# Autodesk Inventor assembly: NewChassis
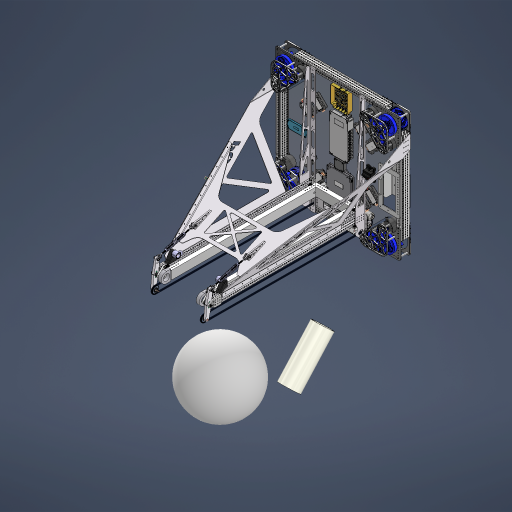
[picture p0: Inventor's stored thumbnail of the model, 512x512]
Saved by Autodesk Inventor 2024.3 (Build 283343000, 343)
## iProperties
ILogicPurgeVersion: 0.0.0.0
OnSaveVersion: 3.5.0.0
OnSaveAssembly: COREAutomationManager
Created: 2025-01-13
Part Number: NewChassis
Document SubType Name: Assembly
Designer: Marcus Tannini
Mfg Approved By: John.Thibert
Mass: 67130.1 g
Surface Area: 92907.1 cm^2
Volume: 47935.8 cm^3
Density: 1.40042 g/cm^3
ModelCat: Uncategorized
CN_MASS: 67.13
Author: Marcus Tannini
## Documents named in this file (43)
- \\clfs\homes\john.thibert\2025-Poseidon-Mechanical\#Poseidon 2025.iam
- \\clfs\homes\john.thibert\2025-Poseidon-Mechanical\ASSY,MK4i,Swerve_Module_INV.iam
- \\clfs\homes\john.thibert\2025-Poseidon-Mechanical\MAXTube-2x1-Holes.ipt
- \\clfs\homes\john.thibert\2025-Poseidon-Mechanical\BellyPanTop.ipt
- \\clfs\homes\john.thibert\2025-Poseidon-Mechanical\BellyPanBot.ipt
- \\clfs\homes\john.thibert\2025-Poseidon-Mechanical\BATTERY,12V.ipt
- \\clfs\homes\john.thibert\2025-Poseidon-Mechanical\CONTROLS,MAIN_BREAKER.ipt
- \\clfs\homes\john.thibert\2025-Poseidon-Mechanical\CONTROLS,MOTOR,NEO,550.ipt
- \\clfs\homes\john.thibert\2025-Poseidon-Mechanical\CONTROLS,PDH.ipt
- \\clfs\homes\john.thibert\2025-Poseidon-Mechanical\CONTROLS,PH.ipt
- \\clfs\homes\john.thibert\2025-Poseidon-Mechanical\CONTROLS,ROBO_RIO.ipt
- \\clfs\homes\john.thibert\2025-Poseidon-Mechanical\CONTROLS,SPARK_MAX.ipt
- \\clfs\homes\john.thibert\2025-Poseidon-Mechanical\CONTROLS,VRM.ipt
- \\clfs\homes\john.thibert\2025-Poseidon-Mechanical\COVER,SPARKMAX.ipt
- \\clfs\homes\john.thibert\2025-Poseidon-Mechanical\ModifiedCase(IncludesPatterning).iam
- \\clfs\homes\john.thibert\2025-Poseidon-Mechanical\PLATE,MOUNT,BATTERY,TOP.ipt
- \\clfs\homes\john.thibert\2025-Poseidon-Mechanical\PLATE,MOUNT,BATTERY,BOT.ipt
- \\clfs\homes\john.thibert\2025-Poseidon-Mechanical\MOUNT,STRAP,BATTERY.ipt
- \\clfs\homes\john.thibert\2025-Poseidon-Mechanical\SPACER,SPROCKET,IDLER,ELEVATOR.ipt
- \\clfs\homes\john.thibert\2025-Poseidon-Mechanical\22.ipt
- \\clfs\homes\john.thibert\2025-Poseidon-Mechanical\PLATE,MOUNT,DRIVE,ELEVATOR.ipt
- \\clfs\homes\john.thibert\2025-Poseidon-Mechanical\PLATE,BEARING,DRIVE,ELEVATOR.ipt
- \\clfs\homes\john.thibert\2025-Poseidon-Mechanical\PURCHASED,HEX_BEARING.ipt
- \\clfs\homes\john.thibert\2025-Poseidon-Mechanical\SHAFT,HEX,0.500in,DRIVE,ELEVATOR.ipt
- \\clfs\homes\john.thibert\2025-Poseidon-Mechanical\PLATE,SIDE,BRACE,RIGHT,ELEVATOR.ipt
- \\clfs\homes\john.thibert\2025-Poseidon-Mechanical\PLATE,SIDE,BRACE,LEFT,ELEVATOR.ipt
- \\clfs\homes\john.thibert\2025-Poseidon-Mechanical\PLATE,TURNBUCKLE,TENSIONER,CHAIN.ipt
- \\clfs\homes\john.thibert\2025-Poseidon-Mechanical\PLATE,BRACE,HORISONTAL,TOP,ELEVATOR.ipt
- \\clfs\homes\john.thibert\2025-Poseidon-Mechanical\TURNBUCKLE,0.25IN_CLEVIS.iam
- \\clfs\homes\john.thibert\2025-Poseidon-Mechanical\STAGE1,ELEVATOR.iam
- \\clfs\homes\john.thibert\2025-Poseidon-Mechanical\ASSY,MAIN,ELEVATOR.iam
- \\clfs\homes\john.thibert\2025-Poseidon-Mechanical\ANGLE,MOUNT,ELEVATOR.ipt
- \\clfs\homes\john.thibert\2025-Poseidon-Mechanical\ANGLE,MOUNT,ELEVATOR,MIRR.ipt
- \\clfs\homes\john.thibert\2025-Poseidon-Mechanical\FABRIC,BUMPERS.ipt
- \\clfs\homes\john.thibert\2025-Poseidon-Mechanical\9293K119_Constant-Force Spring.ipt
- \\clfs\homes\john.thibert\2025-Poseidon-Mechanical\MOUNT,SPRING,ELEVATOR.ipt
- \\clfs\homes\john.thibert\2025-Poseidon-Mechanical\MOUNT,SPRING,ELEVATOR,MIRR.ipt
- \\clfs\homes\john.thibert\2025-Poseidon-Mechanical\VersaPlanetary v2 Dual Stage 10_1 with RS 550 (1).iam
- \\clfs\homes\john.thibert\2025-Poseidon-Mechanical\CORAL.ipt
- \\clfs\homes\john.thibert\2025-Poseidon-Mechanical\algae.ipt
- \\clfs\homes\john.thibert\2025-Poseidon-Mechanical\BRACE,SHAFT,ELEVATOR.ipt
- \\clfs\homes\john.thibert\2025-Poseidon-Mechanical\WCP-0754.ipt
- \\clfs\homes\john.thibert\2025-Poseidon-Mechanical\SPACER,HEX,0.125IN.ipt
## Components (89 placed, 45 different names)
1. FABRIC,BUMPERS.ipt:1 — Flush:323, Mate:335, Mate:336
2. CORAL:1
3. algae:1
4. BellyPanBot.ipt:1 — Mate:66, Mate:353, Mate:354
5. BellyPanTop.ipt:1 — Mate:62, Mate:63, Mate:65, Mate:70, Mate:71, Mate:82, Mate:84, Insert:7, Insert:8, Insert:9, Insert:10, Insert:11, Insert:12, Insert:13, Insert:14, Insert:15, Insert:16, Insert:17, Insert:18, Insert:19, Insert:20, Insert:21, Insert:22, Mate:111, Mate:113, Mate:114, Mate:116, Mate:117, Mate:118, Mate:119, Mate:121, Mate:122, Mate:123, Mate:124, Mate:125, Mate:126, Mate:127, Mate:130, Insert:23, Insert:24, Mate:223, Mate:308, Mate:320, Mate:349, Mate:350
6. MAXTube-2x1-Holes.ipt:1 — Mate:1, Mate:2, Mate:3, Mate:4, Mate:5, Mate:15, Mate:115, Mate:272
7. MAXTube-2x1-Holes.ipt:2 — Mate:6, Mate:7, Mate:8, Mate:9, Mate:10, Mate:11, Mate:62, Mate:309, Mate:310
8. MAXTube-2x1-Holes.ipt:3 — Mate:19, Mate:20, Mate:21, Mate:66, Mate:114, Mate:312, Mate:313, Mate:336
9. MAXTube-2x1-Holes.ipt:4 — Mate:12, Mate:13, Mate:14, Mate:16, Mate:17, Mate:18, Mate:29, Mate:63, Mate:271, Mate:353, Mate:354
10. MOUNT,STRAP,BATTERY.ipt:1 — Mate:357, Mate:358, Mate:359
11. PLATE,MOUNT,BATTERY,BOT.ipt:1 — Mate:320, Mate:321, Mate:351, Mate:352
12. PLATE,MOUNT,BATTERY,TOP.ipt:1 — Mate:127, Mate:349, Mate:350, Mate:351, Mate:352, Mate:356, Mate:357, Mate:358, Mate:359
13. BATTERY,12V.ipt:1 — Mate:321, Mate:356
14. CONTROLS,MAIN_BREAKER.ipt:1 — Mate:82, Mate:111, Mate:116
15. CONTROLS,MOTOR,NEO,550.ipt:1
16. CONTROLS,PDH.ipt:1 — Mate:113, Mate:117, Mate:118, Mate:119
17. CONTROLS,PH.ipt:1 — Insert:23, Insert:24
18. CONTROLS,ROBO_RIO.ipt:1 — Mate:124, Mate:125, Mate:126
19. CONTROLS,SPARK_MAX.ipt:1 — Mate:84, Mate:85, Mate:86, Mate:87
20. CONTROLS,VRM.ipt:1 — Mate:121, Mate:122, Mate:123
21. ModifiedCase(IncludesPatterning).iam:1 [sub-assembly] — Mate:130
22. BRACE,SHAFT,ELEVATOR:1 — Mate:547, Mate:548, Insert:52, Insert:53, Mate:551, Mate:559
23. PURCHASED,HEX_BEARING:3 — Insert:53, Mate:549, Mate:557
24. PURCHASED,HEX_BEARING:4 — Insert:52, Mate:558
25. BRACE,SHAFT,ELEVATOR:2 — Mate:550, Mate:551, Mate:576
26. PURCHASED,HEX_BEARING:5
27. PURCHASED,HEX_BEARING:6 — Mate:555
28. 22:3 — Mate:552, Flush:331, Mate:555, Mate:560
29. WCP-0754:1 — Mate:553, Flush:331
30. SPACER,HEX,0.125IN:1 — Mate:556, Mate:557
31. SPACER,HEX,0.125IN:2 — Mate:558, Mate:559, Mate:560
32. BRACE,SHAFT,ELEVATOR:3 — Mate:565, Mate:568, Mate:569, Mate:576
33. PURCHASED,HEX_BEARING:7 — Mate:575
34. PURCHASED,HEX_BEARING:8
35. BRACE,SHAFT,ELEVATOR:4 — Mate:567, Mate:572, Mate:573
36. PURCHASED,HEX_BEARING:9 — Mate:570, Mate:574
37. PURCHASED,HEX_BEARING:10 — Mate:564
38. 22:4 — Mate:572
39. WCP-0754:2 — Mate:571, Mate:573, Mate:575
40. SPACER,HEX,0.125IN:3 — Mate:569, Mate:570, Mate:571
41. SPACER,HEX,0.125IN:4 — Mate:564, Mate:565
42. 22.ipt:1 — Mate:227, Angle:6
43. 22.ipt:2 — Mate:233, Angle:4, Flush:14
44. 9293K119_Constant-Force Spring:1 — Mate:364, Mate:365
45. 9293K119_Constant-Force Spring:2 — Mate:370, Mate:371
46. ANGLE,MOUNT,ELEVATOR,MIRR.ipt:1 — Mate:308, Mate:309, Mate:310, Mate:311, Mate:312, Mate:313, Mate:314, Mate:315, Flush:329
47. ANGLE,MOUNT,ELEVATOR.ipt:1 — Mate:65, Mate:70, Mate:71, Mate:161, Mate:162, Mate:224, STAGE1 LOWER LIMIT, STAGE1 MIN
48. ASSY,MAIN,ELEVATOR.iam:1 [sub-assembly] — Mate:161, Mate:162, Flush:19, Mate:297, STAGE1 UPPER LIMIT, STAGE1 MAX, Mate:311, Mate:314, Mate:315, Mate:363, Mate:362, Mate:366, Mate:367, Mate:368, Mate:369, Mate:548, Mate:552
49. CONTROLS,MOTOR,NEO,550:3
50. CONTROLS,MOTOR,NEO,550:4
51. MOUNT,SPRING,ELEVATOR,MIRR:1 — Mate:367, Mate:368, Mate:369, Mate:370, Mate:371
52. MOUNT,SPRING,ELEVATOR:1 — Mate:363, Mate:362, Mate:364, Mate:365, Mate:366
53. PLATE,BEARING,DRIVE,ELEVATOR.ipt:1 — Mate:226, Mate:227, Mate:228, Mate:229, Insert:50
54. PLATE,BEARING,DRIVE,ELEVATOR.ipt:2 — Mate:230, Mate:231, Mate:232, Insert:49, Mate:233, Mate:234
55. PLATE,BRACE,HORISONTAL,TOP,ELEVATOR.ipt:1 — Mate:285, Mate:286, Mate:289, Mate:290, Mate:291, Mate:295, Mate:296
56. PLATE,MOUNT,DRIVE,ELEVATOR.ipt:1 — Mate:223, Mate:224, Mate:226, Mate:228, Mate:229, Mate:230, Mate:231, Mate:232, Flush:329, Mate:469, Mate:470, Mate:471, Mate:472, Mate:473, Mate:474
57. PLATE,SIDE,BRACE,LEFT,ELEVATOR.ipt:1 — Mate:271, Mate:289, Mate:290, Mate:291, Mate:335
58. PLATE,SIDE,BRACE,RIGHT,ELEVATOR.ipt:1 — Mate:272
59. PLATE,TURNBUCKLE,TENSIONER,CHAIN.ipt:1 — Mate:285, Mate:296
60. PLATE,TURNBUCKLE,TENSIONER,CHAIN.ipt:2 — Mate:286, Mate:295
61. PURCHASED,HEX_BEARING.ipt:1 — Insert:49, Angle:5
62. PURCHASED,HEX_BEARING.ipt:2 — Insert:50, Angle:7
63. SHAFT,HEX,0.500in,DRIVE,ELEVATOR.ipt:1 — Mate:234, Angle:4, Angle:5, Angle:6, Angle:7, Flush:14
64. SPACER,SPROCKET,IDLER,ELEVATOR.ipt:1
65. SPACER,SPROCKET,IDLER,ELEVATOR.ipt:2
66. STAGE1,ELEVATOR.iam:1 [sub-assembly] — Flush:19, Mate:297, STAGE1 LOWER LIMIT, STAGE1 UPPER LIMIT, STAGE1 MIN, STAGE1 MAX
67. TURNBUCKLE,0.25IN_CLEVIS.iam:1 [sub-assembly]
68. TURNBUCKLE,0.25IN_CLEVIS.iam:2 [sub-assembly]
69. VersaPlanetary v2 Dual Stage 10_1 with RS 550 (1):1 [sub-assembly] — Mate:472, Mate:473, Mate:474, Mate:547, Mate:549, Mate:550, Mate:553, Mate:556
70. VersaPlanetary v2 Dual Stage 10_1 with RS 550 (1):2 [sub-assembly] — Mate:469, Mate:470, Mate:471, Mate:567, Mate:568, Mate:574
71. ASSY,MK4i,Swerve_Module_INV.iam:1 [sub-assembly] — Mate:1, Mate:2, Mate:15
72. ASSY,MK4i,Swerve_Module_INV.iam:2 [sub-assembly] — Mate:3, Mate:4, Mate:5, Mate:6, Mate:7, Mate:8
73. ASSY,MK4i,Swerve_Module_INV.iam:3 [sub-assembly] — Mate:9, Mate:10, Mate:11, Mate:12, Mate:13, Mate:14
74. ASSY,MK4i,Swerve_Module_INV.iam:4 [sub-assembly] — Mate:16, Mate:17, Mate:18, Mate:19, Mate:20, Mate:21, Mate:67
75. CONTROLS,SPARK_MAX.ipt:2
76. CONTROLS,SPARK_MAX.ipt:3
77. CONTROLS,SPARK_MAX.ipt:4
78. CONTROLS,SPARK_MAX.ipt:5
79. CONTROLS,SPARK_MAX.ipt:6
80. CONTROLS,SPARK_MAX.ipt:7
81. CONTROLS,SPARK_MAX.ipt:8
82. COVER,SPARKMAX.ipt:1 — Mate:85, Mate:86, Mate:87, Insert:7, Insert:8
83. COVER,SPARKMAX.ipt:2 — Insert:9, Insert:10
84. COVER,SPARKMAX.ipt:3 — Insert:11, Insert:12
85. COVER,SPARKMAX.ipt:4 — Insert:13, Insert:14
86. COVER,SPARKMAX.ipt:5 — Insert:17, Insert:18
87. COVER,SPARKMAX.ipt:6 — Insert:15, Insert:16
88. COVER,SPARKMAX.ipt:7 — Insert:21, Insert:22
89. COVER,SPARKMAX.ipt:8 — Insert:19, Insert:20
## Relationships (224: Mate 180, Insert 32, Flush 8, Angle 4)
- Mate:1: MAXTube-2x1-Holes.ipt:1 ↔ ASSY,MK4i,Swerve_Module_INV.iam:1
- Mate:2: MAXTube-2x1-Holes.ipt:1 ↔ ASSY,MK4i,Swerve_Module_INV.iam:1
- Mate:3: MAXTube-2x1-Holes.ipt:1 ↔ ASSY,MK4i,Swerve_Module_INV.iam:2
- Mate:4: MAXTube-2x1-Holes.ipt:1 ↔ ASSY,MK4i,Swerve_Module_INV.iam:2
- Mate:5: MAXTube-2x1-Holes.ipt:1 ↔ ASSY,MK4i,Swerve_Module_INV.iam:2
- Mate:6: MAXTube-2x1-Holes.ipt:2 ↔ ASSY,MK4i,Swerve_Module_INV.iam:2
- Mate:7: MAXTube-2x1-Holes.ipt:2 ↔ ASSY,MK4i,Swerve_Module_INV.iam:2
- Mate:8: MAXTube-2x1-Holes.ipt:2 ↔ ASSY,MK4i,Swerve_Module_INV.iam:2
- Mate:9: MAXTube-2x1-Holes.ipt:2 ↔ ASSY,MK4i,Swerve_Module_INV.iam:3
- Mate:10: MAXTube-2x1-Holes.ipt:2 ↔ ASSY,MK4i,Swerve_Module_INV.iam:3
- Mate:11: MAXTube-2x1-Holes.ipt:2 ↔ ASSY,MK4i,Swerve_Module_INV.iam:3
- Mate:12: MAXTube-2x1-Holes.ipt:4 ↔ ASSY,MK4i,Swerve_Module_INV.iam:3
- Mate:13: MAXTube-2x1-Holes.ipt:4 ↔ ASSY,MK4i,Swerve_Module_INV.iam:3
- Mate:14: MAXTube-2x1-Holes.ipt:4 ↔ ASSY,MK4i,Swerve_Module_INV.iam:3
- Mate:15: MAXTube-2x1-Holes.ipt:1 ↔ ASSY,MK4i,Swerve_Module_INV.iam:1
- Mate:16: MAXTube-2x1-Holes.ipt:4 ↔ ASSY,MK4i,Swerve_Module_INV.iam:4
- Mate:17: MAXTube-2x1-Holes.ipt:4 ↔ ASSY,MK4i,Swerve_Module_INV.iam:4
- Mate:18: MAXTube-2x1-Holes.ipt:4 ↔ ASSY,MK4i,Swerve_Module_INV.iam:4
- Mate:19: MAXTube-2x1-Holes.ipt:3 ↔ ASSY,MK4i,Swerve_Module_INV.iam:4
- Mate:20: MAXTube-2x1-Holes.ipt:3 ↔ ASSY,MK4i,Swerve_Module_INV.iam:4
- Mate:21: MAXTube-2x1-Holes.ipt:3 ↔ ASSY,MK4i,Swerve_Module_INV.iam:4
- Mate:29 (-6.35 mm): MAXTube-2x1-Holes.ipt:4
- Mate:62: BellyPanTop.ipt:1 ↔ MAXTube-2x1-Holes.ipt:2
- Mate:63: BellyPanTop.ipt:1 ↔ MAXTube-2x1-Holes.ipt:4
- Mate:65: BellyPanTop.ipt:1 ↔ ANGLE,MOUNT,ELEVATOR.ipt:1
- Mate:66: BellyPanBot.ipt:1 ↔ MAXTube-2x1-Holes.ipt:3
- Mate:67 (35.56 mm): ASSY,MK4i,Swerve_Module_INV.iam:4
- Mate:70: BellyPanTop.ipt:1 ↔ ANGLE,MOUNT,ELEVATOR.ipt:1
- Mate:71: BellyPanTop.ipt:1 ↔ ANGLE,MOUNT,ELEVATOR.ipt:1
- Mate:321: PLATE,MOUNT,BATTERY,BOT.ipt:1 ↔ BATTERY,12V.ipt:1
- Mate:82: BellyPanTop.ipt:1 ↔ CONTROLS,MAIN_BREAKER.ipt:1
- Mate:84: BellyPanTop.ipt:1 ↔ CONTROLS,SPARK_MAX.ipt:1
- Mate:85: CONTROLS,SPARK_MAX.ipt:1 ↔ COVER,SPARKMAX.ipt:1
- Mate:86: CONTROLS,SPARK_MAX.ipt:1 ↔ COVER,SPARKMAX.ipt:1
- Mate:87: CONTROLS,SPARK_MAX.ipt:1 ↔ COVER,SPARKMAX.ipt:1
- Insert:7: BellyPanTop.ipt:1 ↔ COVER,SPARKMAX.ipt:1
- Insert:8: BellyPanTop.ipt:1 ↔ COVER,SPARKMAX.ipt:1
- [Mate]: CONTROLS,SPARK_MAX.ipt:2 ↔ COVER,SPARKMAX.ipt:2
- [Mate]: CONTROLS,SPARK_MAX.ipt:2 ↔ COVER,SPARKMAX.ipt:2
- [Mate]: CONTROLS,SPARK_MAX.ipt:2 ↔ COVER,SPARKMAX.ipt:2
- [Mate]: CONTROLS,SPARK_MAX.ipt:3 ↔ COVER,SPARKMAX.ipt:3
- [Mate]: CONTROLS,SPARK_MAX.ipt:3 ↔ COVER,SPARKMAX.ipt:3
- [Mate]: CONTROLS,SPARK_MAX.ipt:3 ↔ COVER,SPARKMAX.ipt:3
- [Mate]: CONTROLS,SPARK_MAX.ipt:4 ↔ COVER,SPARKMAX.ipt:4
- [Mate]: CONTROLS,SPARK_MAX.ipt:4 ↔ COVER,SPARKMAX.ipt:4
- [Mate]: CONTROLS,SPARK_MAX.ipt:4 ↔ COVER,SPARKMAX.ipt:4
- [Mate]: CONTROLS,SPARK_MAX.ipt:5 ↔ COVER,SPARKMAX.ipt:5
- [Mate]: CONTROLS,SPARK_MAX.ipt:5 ↔ COVER,SPARKMAX.ipt:5
- [Mate]: CONTROLS,SPARK_MAX.ipt:5 ↔ COVER,SPARKMAX.ipt:5
- [Mate]: CONTROLS,SPARK_MAX.ipt:6 ↔ COVER,SPARKMAX.ipt:6
- [Mate]: CONTROLS,SPARK_MAX.ipt:6 ↔ COVER,SPARKMAX.ipt:6
- [Mate]: CONTROLS,SPARK_MAX.ipt:6 ↔ COVER,SPARKMAX.ipt:6
- [Mate]: CONTROLS,SPARK_MAX.ipt:7 ↔ COVER,SPARKMAX.ipt:7
- [Mate]: CONTROLS,SPARK_MAX.ipt:7 ↔ COVER,SPARKMAX.ipt:7
- [Mate]: CONTROLS,SPARK_MAX.ipt:7 ↔ COVER,SPARKMAX.ipt:7
- [Mate]: CONTROLS,SPARK_MAX.ipt:8 ↔ COVER,SPARKMAX.ipt:8
- [Mate]: CONTROLS,SPARK_MAX.ipt:8 ↔ COVER,SPARKMAX.ipt:8
- [Mate]: CONTROLS,SPARK_MAX.ipt:8 ↔ COVER,SPARKMAX.ipt:8
- Insert:9: BellyPanTop.ipt:1 ↔ COVER,SPARKMAX.ipt:2
- Insert:10: BellyPanTop.ipt:1 ↔ COVER,SPARKMAX.ipt:2
- Insert:11: BellyPanTop.ipt:1 ↔ COVER,SPARKMAX.ipt:3
- Insert:12: BellyPanTop.ipt:1 ↔ COVER,SPARKMAX.ipt:3
- Insert:13: BellyPanTop.ipt:1 ↔ COVER,SPARKMAX.ipt:4
- Insert:14: BellyPanTop.ipt:1 ↔ COVER,SPARKMAX.ipt:4
- Insert:15: BellyPanTop.ipt:1 ↔ COVER,SPARKMAX.ipt:6
- Insert:16: BellyPanTop.ipt:1 ↔ COVER,SPARKMAX.ipt:6
- Insert:17: BellyPanTop.ipt:1 ↔ COVER,SPARKMAX.ipt:5
- Insert:18: BellyPanTop.ipt:1 ↔ COVER,SPARKMAX.ipt:5
- Insert:19: BellyPanTop.ipt:1 ↔ COVER,SPARKMAX.ipt:8
- Insert:20: BellyPanTop.ipt:1 ↔ COVER,SPARKMAX.ipt:8
- Insert:21: BellyPanTop.ipt:1 ↔ COVER,SPARKMAX.ipt:7
- Insert:22: BellyPanTop.ipt:1 ↔ COVER,SPARKMAX.ipt:7
- Mate:111: BellyPanTop.ipt:1 ↔ CONTROLS,MAIN_BREAKER.ipt:1
- Mate:113: BellyPanTop.ipt:1 ↔ CONTROLS,PDH.ipt:1
- Mate:114: BellyPanTop.ipt:1 ↔ MAXTube-2x1-Holes.ipt:3
- Mate:115 (-374.65 mm): MAXTube-2x1-Holes.ipt:1
- Mate:116 (0.254 mm): BellyPanTop.ipt:1 ↔ CONTROLS,MAIN_BREAKER.ipt:1
- Mate:117: BellyPanTop.ipt:1 ↔ CONTROLS,PDH.ipt:1
- Mate:118: BellyPanTop.ipt:1 ↔ CONTROLS,PDH.ipt:1
- Mate:119: BellyPanTop.ipt:1 ↔ CONTROLS,PDH.ipt:1
- Mate:121: BellyPanTop.ipt:1 ↔ CONTROLS,VRM.ipt:1
- Mate:122: BellyPanTop.ipt:1 ↔ CONTROLS,VRM.ipt:1
- Mate:123: BellyPanTop.ipt:1 ↔ CONTROLS,VRM.ipt:1
- Mate:124: BellyPanTop.ipt:1 ↔ CONTROLS,ROBO_RIO.ipt:1
- Mate:125: BellyPanTop.ipt:1 ↔ CONTROLS,ROBO_RIO.ipt:1
- Mate:126: BellyPanTop.ipt:1 ↔ CONTROLS,ROBO_RIO.ipt:1
- Mate:127: BellyPanTop.ipt:1 ↔ PLATE,MOUNT,BATTERY,TOP.ipt:1
- Mate:130: BellyPanTop.ipt:1 ↔ ModifiedCase(IncludesPatterning).iam:1
- Insert:23: BellyPanTop.ipt:1 ↔ CONTROLS,PH.ipt:1
- Insert:24: BellyPanTop.ipt:1 ↔ CONTROLS,PH.ipt:1
- Mate:161: ANGLE,MOUNT,ELEVATOR.ipt:1 ↔ ASSY,MAIN,ELEVATOR.iam:1
- Mate:162: ANGLE,MOUNT,ELEVATOR.ipt:1 ↔ ASSY,MAIN,ELEVATOR.iam:1
- [Mate]: ANGLE,MOUNT,ELEVATOR.ipt:1 ↔ ASSY,MAIN,ELEVATOR.iam:1
- [Insert]: ASSY,MAIN,ELEVATOR.iam:1 ↔ SPACER,SPROCKET,IDLER,ELEVATOR.ipt:1
- [Insert]: ASSY,MAIN,ELEVATOR.iam:1 ↔ SPACER,SPROCKET,IDLER,ELEVATOR.ipt:1
- [Flush]: 22.ipt:1 ↔ ASSY,MAIN,ELEVATOR.iam:1
- [Insert]: ASSY,MAIN,ELEVATOR.iam:1 ↔ SPACER,SPROCKET,IDLER,ELEVATOR.ipt:2
- [Insert]: ASSY,MAIN,ELEVATOR.iam:1 ↔ SPACER,SPROCKET,IDLER,ELEVATOR.ipt:2
- Mate:223: BellyPanTop.ipt:1 ↔ PLATE,MOUNT,DRIVE,ELEVATOR.ipt:1
- Mate:224: ANGLE,MOUNT,ELEVATOR.ipt:1 ↔ PLATE,MOUNT,DRIVE,ELEVATOR.ipt:1
- Mate:226: PLATE,BEARING,DRIVE,ELEVATOR.ipt:1 ↔ PLATE,MOUNT,DRIVE,ELEVATOR.ipt:1
- Mate:227: 22.ipt:1 ↔ PLATE,BEARING,DRIVE,ELEVATOR.ipt:1
- Mate:228: PLATE,BEARING,DRIVE,ELEVATOR.ipt:1 ↔ PLATE,MOUNT,DRIVE,ELEVATOR.ipt:1
- Mate:229: PLATE,BEARING,DRIVE,ELEVATOR.ipt:1 ↔ PLATE,MOUNT,DRIVE,ELEVATOR.ipt:1
- Mate:230: PLATE,BEARING,DRIVE,ELEVATOR.ipt:2 ↔ PLATE,MOUNT,DRIVE,ELEVATOR.ipt:1
- Mate:231: PLATE,BEARING,DRIVE,ELEVATOR.ipt:2 ↔ PLATE,MOUNT,DRIVE,ELEVATOR.ipt:1
- Mate:232: PLATE,BEARING,DRIVE,ELEVATOR.ipt:2 ↔ PLATE,MOUNT,DRIVE,ELEVATOR.ipt:1
- Insert:49: PLATE,BEARING,DRIVE,ELEVATOR.ipt:2 ↔ PURCHASED,HEX_BEARING.ipt:1
- Insert:50: PLATE,BEARING,DRIVE,ELEVATOR.ipt:1 ↔ PURCHASED,HEX_BEARING.ipt:2
- Mate:233: 22.ipt:2 ↔ PLATE,BEARING,DRIVE,ELEVATOR.ipt:2
- Mate:234: PLATE,BEARING,DRIVE,ELEVATOR.ipt:2 ↔ SHAFT,HEX,0.500in,DRIVE,ELEVATOR.ipt:1
- Angle:4 (0 deg): 22.ipt:2 ↔ SHAFT,HEX,0.500in,DRIVE,ELEVATOR.ipt:1
- Angle:5 (0 deg): PURCHASED,HEX_BEARING.ipt:1 ↔ SHAFT,HEX,0.500in,DRIVE,ELEVATOR.ipt:1
- Angle:6 (0 deg): 22.ipt:1 ↔ SHAFT,HEX,0.500in,DRIVE,ELEVATOR.ipt:1
- Angle:7 (0 deg): PURCHASED,HEX_BEARING.ipt:2 ↔ SHAFT,HEX,0.500in,DRIVE,ELEVATOR.ipt:1
- [Flush]: 22.ipt:2 ↔ ASSY,MAIN,ELEVATOR.iam:1
- [Mate]: ASSY,MAIN,ELEVATOR.iam:1 ↔ PLATE,SIDE,BRACE,LEFT,ELEVATOR.ipt:1
- [Mate]: ASSY,MAIN,ELEVATOR.iam:1 ↔ PLATE,SIDE,BRACE,LEFT,ELEVATOR.ipt:1
- [Mate]: 22.ipt:1 ↔ ASSY,MAIN,ELEVATOR.iam:1
- Flush:14 (-15.875 mm): 22.ipt:2 ↔ SHAFT,HEX,0.500in,DRIVE,ELEVATOR.ipt:1
- [Mate]: ASSY,MAIN,ELEVATOR.iam:1 ↔ PLATE,SIDE,BRACE,LEFT,ELEVATOR.ipt:1
- [Mate]: ASSY,MAIN,ELEVATOR.iam:1 ↔ PLATE,SIDE,BRACE,RIGHT,ELEVATOR.ipt:1
- [Mate]: ASSY,MAIN,ELEVATOR.iam:1 ↔ PLATE,SIDE,BRACE,RIGHT,ELEVATOR.ipt:1
- [Mate]: ASSY,MAIN,ELEVATOR.iam:1 ↔ PLATE,SIDE,BRACE,RIGHT,ELEVATOR.ipt:1
- Mate:271: MAXTube-2x1-Holes.ipt:4 ↔ PLATE,SIDE,BRACE,LEFT,ELEVATOR.ipt:1
- Mate:272: MAXTube-2x1-Holes.ipt:1 ↔ PLATE,SIDE,BRACE,RIGHT,ELEVATOR.ipt:1
- [Mate]: ASSY,MAIN,ELEVATOR.iam:1 ↔ TURNBUCKLE,0.25IN_CLEVIS.iam:1
- [Mate]: ASSY,MAIN,ELEVATOR.iam:1 ↔ TURNBUCKLE,0.25IN_CLEVIS.iam:1
- [Mate]: ASSY,MAIN,ELEVATOR.iam:1 ↔ TURNBUCKLE,0.25IN_CLEVIS.iam:2
- [Mate]: ASSY,MAIN,ELEVATOR.iam:1 ↔ TURNBUCKLE,0.25IN_CLEVIS.iam:2
- Mate:285: PLATE,BRACE,HORISONTAL,TOP,ELEVATOR.ipt:1 ↔ PLATE,TURNBUCKLE,TENSIONER,CHAIN.ipt:1
- Mate:286: PLATE,BRACE,HORISONTAL,TOP,ELEVATOR.ipt:1 ↔ PLATE,TURNBUCKLE,TENSIONER,CHAIN.ipt:2
- Mate:289: PLATE,BRACE,HORISONTAL,TOP,ELEVATOR.ipt:1 ↔ PLATE,SIDE,BRACE,LEFT,ELEVATOR.ipt:1
- Mate:290: PLATE,BRACE,HORISONTAL,TOP,ELEVATOR.ipt:1 ↔ PLATE,SIDE,BRACE,LEFT,ELEVATOR.ipt:1
- Mate:291: PLATE,BRACE,HORISONTAL,TOP,ELEVATOR.ipt:1 ↔ PLATE,SIDE,BRACE,LEFT,ELEVATOR.ipt:1
- [Mate]: 22.ipt:2 ↔ ASSY,MAIN,ELEVATOR.iam:1
- Mate:295: PLATE,BRACE,HORISONTAL,TOP,ELEVATOR.ipt:1 ↔ PLATE,TURNBUCKLE,TENSIONER,CHAIN.ipt:2
- Mate:296: PLATE,BRACE,HORISONTAL,TOP,ELEVATOR.ipt:1 ↔ PLATE,TURNBUCKLE,TENSIONER,CHAIN.ipt:1
- Flush:19: ASSY,MAIN,ELEVATOR.iam:1 ↔ STAGE1,ELEVATOR.iam:1
- Mate:297: ASSY,MAIN,ELEVATOR.iam:1 ↔ STAGE1,ELEVATOR.iam:1
- STAGE1 LOWER LIMIT [Mate]: ANGLE,MOUNT,ELEVATOR.ipt:1 ↔ STAGE1,ELEVATOR.iam:1
- STAGE1 UPPER LIMIT [Mate]: ASSY,MAIN,ELEVATOR.iam:1 ↔ STAGE1,ELEVATOR.iam:1
- STAGE1 MIN [Mate]: ANGLE,MOUNT,ELEVATOR.ipt:1 ↔ STAGE1,ELEVATOR.iam:1
- STAGE1 MAX [Mate] (3.175 mm): ASSY,MAIN,ELEVATOR.iam:1 ↔ STAGE1,ELEVATOR.iam:1
- Mate:308: BellyPanTop.ipt:1 ↔ ANGLE,MOUNT,ELEVATOR,MIRR.ipt:1
- Mate:309: MAXTube-2x1-Holes.ipt:2 ↔ ANGLE,MOUNT,ELEVATOR,MIRR.ipt:1
- Mate:310: MAXTube-2x1-Holes.ipt:2 ↔ ANGLE,MOUNT,ELEVATOR,MIRR.ipt:1
- Mate:311: ANGLE,MOUNT,ELEVATOR,MIRR.ipt:1 ↔ ASSY,MAIN,ELEVATOR.iam:1
- Mate:312: MAXTube-2x1-Holes.ipt:3 ↔ ANGLE,MOUNT,ELEVATOR,MIRR.ipt:1
- Mate:313: MAXTube-2x1-Holes.ipt:3 ↔ ANGLE,MOUNT,ELEVATOR,MIRR.ipt:1
- Mate:314: ANGLE,MOUNT,ELEVATOR,MIRR.ipt:1 ↔ ASSY,MAIN,ELEVATOR.iam:1
- Mate:315: ANGLE,MOUNT,ELEVATOR,MIRR.ipt:1 ↔ ASSY,MAIN,ELEVATOR.iam:1
- Mate:320: BellyPanTop.ipt:1 ↔ PLATE,MOUNT,BATTERY,BOT.ipt:1
- Flush:323 (146.05 mm): FABRIC,BUMPERS.ipt:1
- Mate:335 (3.175 mm): FABRIC,BUMPERS.ipt:1 ↔ PLATE,SIDE,BRACE,LEFT,ELEVATOR.ipt:1
- Mate:336 (6.35 mm): FABRIC,BUMPERS.ipt:1 ↔ MAXTube-2x1-Holes.ipt:3
- Mate:349: BellyPanTop.ipt:1 ↔ PLATE,MOUNT,BATTERY,TOP.ipt:1
- Mate:350: BellyPanTop.ipt:1 ↔ PLATE,MOUNT,BATTERY,TOP.ipt:1
- Mate:351: PLATE,MOUNT,BATTERY,BOT.ipt:1 ↔ PLATE,MOUNT,BATTERY,TOP.ipt:1
- Mate:352: PLATE,MOUNT,BATTERY,BOT.ipt:1 ↔ PLATE,MOUNT,BATTERY,TOP.ipt:1
- Mate:353: BellyPanBot.ipt:1 ↔ MAXTube-2x1-Holes.ipt:4
- Mate:354: BellyPanBot.ipt:1 ↔ MAXTube-2x1-Holes.ipt:4
- Mate:356 (19.05 mm): PLATE,MOUNT,BATTERY,TOP.ipt:1 ↔ BATTERY,12V.ipt:1
- Mate:357: MOUNT,STRAP,BATTERY.ipt:1 ↔ PLATE,MOUNT,BATTERY,TOP.ipt:1
- Mate:358: MOUNT,STRAP,BATTERY.ipt:1 ↔ PLATE,MOUNT,BATTERY,TOP.ipt:1
- Mate:359: MOUNT,STRAP,BATTERY.ipt:1 ↔ PLATE,MOUNT,BATTERY,TOP.ipt:1
- Mate:363: ASSY,MAIN,ELEVATOR.iam:1 ↔ MOUNT,SPRING,ELEVATOR:1
- Mate:362: ASSY,MAIN,ELEVATOR.iam:1 ↔ MOUNT,SPRING,ELEVATOR:1
- Mate:364: 9293K119_Constant-Force Spring:1 ↔ MOUNT,SPRING,ELEVATOR:1
- Mate:365 (1.5875 mm): 9293K119_Constant-Force Spring:1 ↔ MOUNT,SPRING,ELEVATOR:1
- Mate:366: ASSY,MAIN,ELEVATOR.iam:1 ↔ MOUNT,SPRING,ELEVATOR:1
- Mate:367: ASSY,MAIN,ELEVATOR.iam:1 ↔ MOUNT,SPRING,ELEVATOR,MIRR:1
- Mate:368: ASSY,MAIN,ELEVATOR.iam:1 ↔ MOUNT,SPRING,ELEVATOR,MIRR:1
- Mate:369: ASSY,MAIN,ELEVATOR.iam:1 ↔ MOUNT,SPRING,ELEVATOR,MIRR:1
- Mate:370: 9293K119_Constant-Force Spring:2 ↔ MOUNT,SPRING,ELEVATOR,MIRR:1
- Mate:371 (1.5875 mm): 9293K119_Constant-Force Spring:2 ↔ MOUNT,SPRING,ELEVATOR,MIRR:1
- Flush:329: ANGLE,MOUNT,ELEVATOR,MIRR.ipt:1 ↔ PLATE,MOUNT,DRIVE,ELEVATOR.ipt:1
- [Mate]: CONTROLS,MOTOR,NEO,550:3 ↔ VersaPlanetary v2 Dual Stage 10_1 with RS 550 (1):1
- [Mate]: CONTROLS,MOTOR,NEO,550:3 ↔ VersaPlanetary v2 Dual Stage 10_1 with RS 550 (1):1
- [Mate]: CONTROLS,MOTOR,NEO,550:4 ↔ VersaPlanetary v2 Dual Stage 10_1 with RS 550 (1):2
- [Mate]: CONTROLS,MOTOR,NEO,550:4 ↔ VersaPlanetary v2 Dual Stage 10_1 with RS 550 (1):2
- Mate:469: PLATE,MOUNT,DRIVE,ELEVATOR.ipt:1 ↔ VersaPlanetary v2 Dual Stage 10_1 with RS 550 (1):2
- Mate:470: PLATE,MOUNT,DRIVE,ELEVATOR.ipt:1 ↔ VersaPlanetary v2 Dual Stage 10_1 with RS 550 (1):2
- Mate:471: PLATE,MOUNT,DRIVE,ELEVATOR.ipt:1 ↔ VersaPlanetary v2 Dual Stage 10_1 with RS 550 (1):2
- Mate:472: PLATE,MOUNT,DRIVE,ELEVATOR.ipt:1 ↔ VersaPlanetary v2 Dual Stage 10_1 with RS 550 (1):1
- Mate:473: PLATE,MOUNT,DRIVE,ELEVATOR.ipt:1 ↔ VersaPlanetary v2 Dual Stage 10_1 with RS 550 (1):1
- Mate:474: PLATE,MOUNT,DRIVE,ELEVATOR.ipt:1 ↔ VersaPlanetary v2 Dual Stage 10_1 with RS 550 (1):1
- Mate:547: BRACE,SHAFT,ELEVATOR:1 ↔ VersaPlanetary v2 Dual Stage 10_1 with RS 550 (1):1
- Mate:548 (0.254 mm): BRACE,SHAFT,ELEVATOR:1 ↔ ASSY,MAIN,ELEVATOR.iam:1
- Insert:52: BRACE,SHAFT,ELEVATOR:1 ↔ PURCHASED,HEX_BEARING:4
- Insert:53: BRACE,SHAFT,ELEVATOR:1 ↔ PURCHASED,HEX_BEARING:3
- Mate:549: PURCHASED,HEX_BEARING:3 ↔ VersaPlanetary v2 Dual Stage 10_1 with RS 550 (1):1
- [Insert]: BRACE,SHAFT,ELEVATOR:2 ↔ PURCHASED,HEX_BEARING:6
- [Insert]: BRACE,SHAFT,ELEVATOR:2 ↔ PURCHASED,HEX_BEARING:5
- Mate:550: BRACE,SHAFT,ELEVATOR:2 ↔ VersaPlanetary v2 Dual Stage 10_1 with RS 550 (1):1
- Mate:551: BRACE,SHAFT,ELEVATOR:1 ↔ BRACE,SHAFT,ELEVATOR:2
- Mate:552: 22:3 ↔ ASSY,MAIN,ELEVATOR.iam:1
- Mate:553: WCP-0754:1 ↔ VersaPlanetary v2 Dual Stage 10_1 with RS 550 (1):1
- Flush:331: 22:3 ↔ WCP-0754:1
- Mate:555: PURCHASED,HEX_BEARING:6 ↔ 22:3
- Mate:556: SPACER,HEX,0.125IN:1 ↔ VersaPlanetary v2 Dual Stage 10_1 with RS 550 (1):1
- Mate:557: PURCHASED,HEX_BEARING:3 ↔ SPACER,HEX,0.125IN:1
- Mate:558: PURCHASED,HEX_BEARING:4 ↔ SPACER,HEX,0.125IN:2
- Mate:559: BRACE,SHAFT,ELEVATOR:1 ↔ SPACER,HEX,0.125IN:2
- Mate:560: 22:3 ↔ SPACER,HEX,0.125IN:2
- [Insert]: BRACE,SHAFT,ELEVATOR:3 ↔ PURCHASED,HEX_BEARING:8
- [Insert]: BRACE,SHAFT,ELEVATOR:3 ↔ PURCHASED,HEX_BEARING:7
- [Insert]: BRACE,SHAFT,ELEVATOR:4 ↔ PURCHASED,HEX_BEARING:10
- [Insert]: BRACE,SHAFT,ELEVATOR:4 ↔ PURCHASED,HEX_BEARING:9
- [Mate]: BRACE,SHAFT,ELEVATOR:3 ↔ BRACE,SHAFT,ELEVATOR:4
- [Flush]: 22:4 ↔ WCP-0754:2
- Mate:564: PURCHASED,HEX_BEARING:10 ↔ SPACER,HEX,0.125IN:4
- Mate:565: BRACE,SHAFT,ELEVATOR:3 ↔ SPACER,HEX,0.125IN:4
- [Mate]: 22:4 ↔ SPACER,HEX,0.125IN:4
- Mate:567: BRACE,SHAFT,ELEVATOR:4 ↔ VersaPlanetary v2 Dual Stage 10_1 with RS 550 (1):2
- Mate:568: BRACE,SHAFT,ELEVATOR:3 ↔ VersaPlanetary v2 Dual Stage 10_1 with RS 550 (1):2
- Mate:569: BRACE,SHAFT,ELEVATOR:3 ↔ SPACER,HEX,0.125IN:3
- Mate:570: PURCHASED,HEX_BEARING:9 ↔ SPACER,HEX,0.125IN:3
- Mate:571: WCP-0754:2 ↔ SPACER,HEX,0.125IN:3
- Mate:572: BRACE,SHAFT,ELEVATOR:4 ↔ 22:4
- Mate:573: BRACE,SHAFT,ELEVATOR:4 ↔ WCP-0754:2
- Mate:574: PURCHASED,HEX_BEARING:9 ↔ VersaPlanetary v2 Dual Stage 10_1 with RS 550 (1):2
- Mate:575: PURCHASED,HEX_BEARING:7 ↔ WCP-0754:2
- Mate:576: BRACE,SHAFT,ELEVATOR:2 ↔ BRACE,SHAFT,ELEVATOR:3
## Named parameters: d160_d155 = 0 mm, d161_d156 = 0 mm, d162_d157 = 0 mm, d163_d155 = 0 mm, d164_d156 = 0 mm, d165_d157 = 0 mm, d166_d155 = 0 mm, d167_d156 = 0 mm, d168_d157 = 0 mm, d169_d155 = 0 mm, d170_d156 = 0 mm, d171_d157 = 0 mm, d172_d155 = 0 mm, d173_d156 = 0 mm, d174_d157 = 0 mm, d175_d155 = 0 mm, d176_d156 = 0 mm, d177_d157 = 0 mm, d178_d155 = 0 mm, d179_d156 = 0 mm, d180_d157 = 0 mm, d518_d513 = 0 mm, d875_d873 = 0 mm, d876_d874 = 0 mm, d967_d875_d873 = 0 mm, d968_d876_d874 = 0 mm, d1116_d1113 = 0 mm, d1117_d1114 = 0 mm, d1135_d1113 = 0 mm, d1136_d1114 = 0 mm, d1137_d1116_d1113 = 0 mm, d1138_d1117_d1114 = 0 mm, d1139_d1123 = 0 mm, d1140_d1127 = 0 mm, d1143_d1132 = 0 mm, d1144_d1133 = 0 mm, d1145_d1134 = 0 mm
